# Autodesk Inventor assembly: гроб для задницы цел_MIR1_MIR
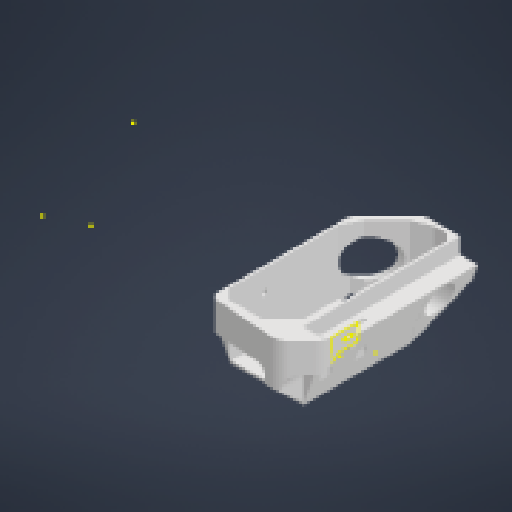
[picture p0: Inventor's stored thumbnail of the model, 512x512]
Saved by Autodesk Inventor 2025 (Build 290162000, 162)
## iProperties
Created: 2024-08-15
Part Number: гроб для задницы цел_MIR1_MIR
Document SubType Name: Assembly
Designer: GameHD
Author: GameHD
## Documents named in this file (3)
- C:\Users\GameHD\Desktop\робототехника\гроб для задницы цел_MIR1_MIR.iam
- C:\Users\GameHD\Desktop\робототехника\гроб для задницы_MIR1_MIR.ipt
- C:\Users\GameHD\Desktop\робототехника\гроб для задницы 2 ч_MIR1_MIR.ipt
## Components (2 placed, 2 different names)
1. гроб для задницы_MIR1_MIR:1 — Жесткий:1
2. гроб для задницы 2 ч_MIR1_MIR:1 — Жесткий:1
## Relationships (1: WeldJoint 1)
- Жесткий:1 [WeldJoint]: гроб для задницы_MIR1_MIR:1 ↔ гроб для задницы 2 ч_MIR1_MIR:1
